# Autodesk Inventor assembly: hblsd_assembly
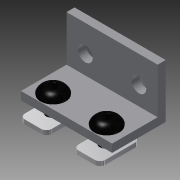
[picture p0: Inventor's stored thumbnail of the model, 180x180]
Saved by Autodesk Inventor 2014 (Build 180170000, 170)
## iProperties
Created: 2013-05-29
Part Number: hblsd_assembly
Document SubType Name: Assembly
Designer: Edward
Author: Edward
## Documents named in this file (4)
- C:\Users\Edward\Desktop\Shapeoko_v2.0\hblsd_assembly.iam
- C:\Users\Edward\Desktop\Shapeoko_v2.0\HNKK55.ipt
- C:\Users\Edward\Desktop\Shapeoko_v2.0\hblsd5_2_03.ipt
- C:\Users\Edward\Desktop\Shapeoko_v2.0\91239A222.ipt
## Components (5 placed, 3 different names)
1. HNKK55:3 — Insert:5, Angle:2
2. HNKK55:4 — Insert:6, Angle:1
3. hblsd5_2_03:1 — Insert:3, Insert:4, Insert:5, Insert:6, Angle:1, Angle:2
4. 91239A222:2 — Insert:4
5. 91239A222:4 — Insert:3
## Relationships (6: Insert 4, Angle 2)
- Insert:3: hblsd5_2_03:1 ↔ 91239A222:4
- Insert:4: hblsd5_2_03:1 ↔ 91239A222:2
- Insert:5 (3 mm): HNKK55:3 ↔ hblsd5_2_03:1
- Insert:6 (3 mm): HNKK55:4 ↔ hblsd5_2_03:1
- Angle:1 (0 deg): HNKK55:4 ↔ hblsd5_2_03:1
- Angle:2 (0 deg): HNKK55:3 ↔ hblsd5_2_03:1
